# Autodesk Inventor assembly: mould_top_p2
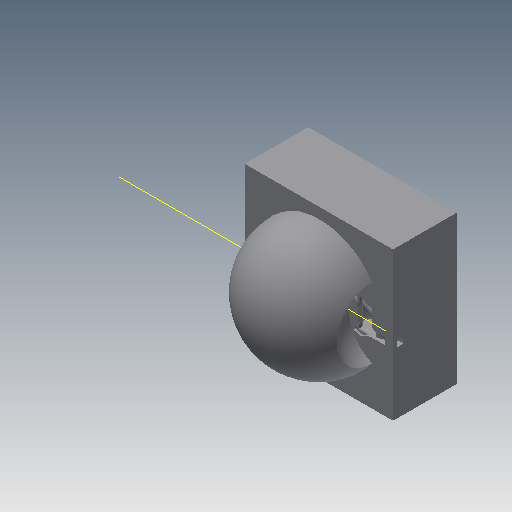
[picture p0: Inventor's stored thumbnail of the model, 512x512]
Saved by Autodesk Inventor 2017 (Build 210142000, 142)
## iProperties
Created: 2018-06-07
Part Number: mould_top_p2
Document SubType Name: Assembly
Designer: Nic
Author: Nic
## Documents named in this file (3)
- C:\Users\Nic\Documents\Antenna\mould_top_p2.iam
- C:\Users\Nic\Documents\Antenna\mould_top_proc1.ipt
- C:\Users\Nic\Documents\Antenna\sensor_pad.ipt
## Components (2 placed, 2 different names)
1. mould_top_proc1:1 — Ball:1, Mate:2, Mate:3, Mate:4
2. sensor_pad:1 — Ball:1, Mate:1
## Relationships (5: Mate 4, BallJoint 1)
- Ball:1: mould_top_proc1:1 ↔ sensor_pad:1
- Mate:1: sensor_pad:1
- Mate:2: mould_top_proc1:1
- Mate:3: mould_top_proc1:1
- Mate:4: mould_top_proc1:1
